# Autodesk Inventor assembly: RPi Zero
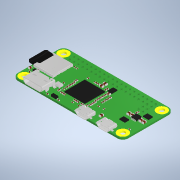
[picture p0: Inventor's stored thumbnail of the model, 180x180]
Saved by Autodesk Inventor 2020.3 (Build 243373010, 373A)
## iProperties
Created: 2016-07-22
Part Number: RPi Zero
Description: STEP AP203
Document SubType Name: Assembly
Designer: Michael
Sending System: SolidWorks 2013
Preprocessor: SwSTEP 2.0
Title: RapberryPiZero.STEP
Revision Number: ANY
## Documents named in this file (17)
- C:\Users\Michael\Dropbox (MIT)\College\Work\CSAIL HCIE UROP\CAD Files\Phone Case\RPi Zero\RPi Zero.iam
- C:\Users\Michael\Dropbox (MIT)\College\Work\CSAIL HCIE UROP\CAD Files\Phone Case\RPi Zero\Raspberry_pizero_PCB.ipt
- C:\Users\Michael\Dropbox (MIT)\College\Work\CSAIL HCIE UROP\CAD Files\Phone Case\RPi Zero\Micro USB_input_female (short)-SMT.ipt
- C:\Users\Michael\Dropbox (MIT)\College\Work\CSAIL HCIE UROP\CAD Files\Phone Case\RPi Zero\0204 - Capacitor.ipt
- C:\Users\Michael\Dropbox (MIT)\College\Work\CSAIL HCIE UROP\CAD Files\Phone Case\RPi Zero\0204- Resistor.ipt
- C:\Users\Michael\Dropbox (MIT)\College\Work\CSAIL HCIE UROP\CAD Files\Phone Case\RPi Zero\CAP-0306.ipt
- C:\Users\Michael\Dropbox (MIT)\College\Work\CSAIL HCIE UROP\CAD Files\Phone Case\RPi Zero\Raspberry_pizero_BCM2835 with VC4.ipt
- C:\Users\Michael\Dropbox (MIT)\College\Work\CSAIL HCIE UROP\CAD Files\Phone Case\RPi Zero\Crystal 3.4x2.4mm.ipt
- C:\Users\Michael\Dropbox (MIT)\College\Work\CSAIL HCIE UROP\CAD Files\Phone Case\RPi Zero\32,768 Khz Crystal.ipt
- C:\Users\Michael\Dropbox (MIT)\College\Work\CSAIL HCIE UROP\CAD Files\Phone Case\RPi Zero\0805- Capacitor.ipt
- C:\Users\Michael\Dropbox (MIT)\College\Work\CSAIL HCIE UROP\CAD Files\Phone Case\RPi Zero\0204 - Capacitor Brown.ipt
- C:\Users\Michael\Dropbox (MIT)\College\Work\CSAIL HCIE UROP\CAD Files\Phone Case\RPi Zero\6-Pin SOT.ipt
- C:\Users\Michael\Dropbox (MIT)\College\Work\CSAIL HCIE UROP\CAD Files\Phone Case\RPi Zero\micro sd molex.ipt
- C:\Users\Michael\Dropbox (MIT)\College\Work\CSAIL HCIE UROP\CAD Files\Phone Case\RPi Zero\hdmi type C.ipt
- C:\Users\Michael\Dropbox (MIT)\College\Work\CSAIL HCIE UROP\CAD Files\Phone Case\RPi Zero\Voltage Regulator 3x3mm 12-Pin.ipt
- C:\Users\Michael\Dropbox (MIT)\College\Work\CSAIL HCIE UROP\CAD Files\Phone Case\RPi Zero\1210 inductor.ipt
- C:\Users\Michael\Dropbox\College\Work\CSAIL HCIE UROP\CAD Files\Phone Case\RPi Zero\Micro SD Card.ipt
## Components (82 placed, 82 different names)
1. Raspberry_pizero_PCB_1
2. Micro USB_input_female (short)-SMT_2
3. Micro USB_input_female (short)-SMT_3
4. 0204 - Capacitor_4
5. 0204 - Capacitor_5
6. 0204 - Capacitor_6
7. 0204 - Capacitor_7
8. 0204 - Capacitor_8
9. 0204 - Capacitor_9
10. 0204 - Capacitor_10
11. 0204 - Capacitor_11
12. 0204 - Capacitor_12
13. 0204 - Capacitor_13
14. 0204 - Capacitor_14
15. 0204 - Capacitor_15
16. 0204 - Capacitor_16
17. 0204 - Capacitor_17
18. 0204 - Capacitor_18
19. 0204 - Capacitor_19
20. 0204 - Capacitor_20
21. 0204 - Capacitor_21
22. 0204 - Capacitor_22
23. 0204 - Capacitor_23
24. 0204 - Capacitor_24
25. 0204 - Capacitor_25
26. 0204 - Capacitor_26
27. 0204 - Capacitor_27
28. 0204 - Capacitor_28
29. 0204 - Capacitor_29
30. 0204 - Capacitor_30
31. 0204 - Capacitor_31
32. 0204 - Capacitor_32
33. 0204 - Capacitor_33
34. 0204 - Capacitor_34
35. 0204 - Capacitor_35
36. 0204- Resistor_36
37. 0204- Resistor_37
38. 0204- Resistor_38
39. 0204- Resistor_39
40. 0204- Resistor_40
41. 0204- Resistor_41
42. 0204- Resistor_42
43. 0204- Resistor_43
44. 0204- Resistor_44
45. 0204- Resistor_45
46. 0204- Resistor_46
47. CAP-0306_47
48. CAP-0306_48
49. Raspberry_pizero_BCM2835 with VC4_49
50. Crystal 3.4x2.4mm_50
51. 0204- Resistor_51
52. 0204- Resistor_52
53. 0204- Resistor_53
54. 32,768 Khz Crystal_54
55. 0805- Capacitor_55
56. 0805- Capacitor_56
57. 0805- Capacitor_57
58. 0805- Capacitor_58
59. 0805- Capacitor_59
60. 0805- Capacitor_60
61. 0805- Capacitor_61
62. 0204- Resistor_62
63. 0204- Resistor_63
64. 0204 - Capacitor_64
65. 0204 - Capacitor Brown_65
66. 0204 - Capacitor Brown_66
67. 0204 - Capacitor Brown_67
68. 0204 - Capacitor Brown_68
69. 0204 - Capacitor Brown_69
70. 0204 - Capacitor Brown_70
71. 0204 - Capacitor Brown_71
72. 0204 - Capacitor Brown_72
73. 0204- Resistor_73
74. 6-Pin SOT_74
75. micro sd molex_75 — Mate:1, Mate:2, Mate:3
76. hdmi type C_76
77. Voltage Regulator 3x3mm 12-Pin_77
78. 1210 inductor_78
79. 1210 inductor_79
80. 1210 inductor_80
81. 0204 - Capacitor_81
82. Micro SD Card:1 — Mate:1, Mate:2, Mate:3
## Relationships (3: Mate 3)
- Mate:1: micro sd molex_75 ↔ Micro SD Card:1
- Mate:2: micro sd molex_75 ↔ Micro SD Card:1
- Mate:3 (-15.5 mm): micro sd molex_75 ↔ Micro SD Card:1
